# Autodesk Inventor assembly: Assembly
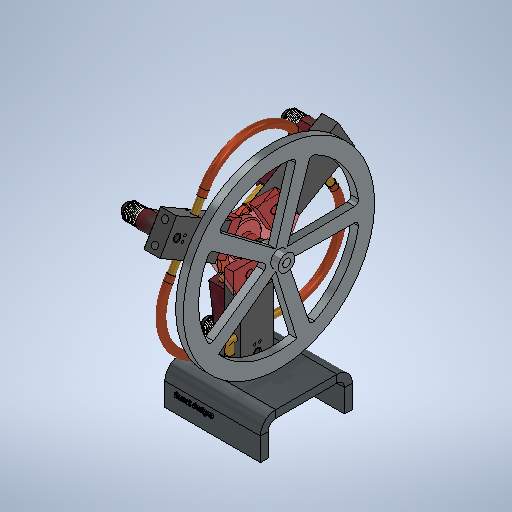
[picture p0: Inventor's stored thumbnail of the model, 512x512]
Saved by Autodesk Inventor 2025 (Build 290162010, 162A)
## iProperties
Created: 2024-06-06
Part Number: Assembly
Document SubType Name: Assembly
Designer: ffogue
Author: ffogue
## Documents named in this file (16)
- C:\Users\Fabri\Documents\Inventor\oscillatingEngine\Assembly.iam
- C:\Users\Fabri\Documents\Inventor\oscillatingEngine\support.ipt
- C:\Users\Fabri\Documents\Inventor\oscillatingEngine\base.ipt
- C:\Users\Fabri\Documents\Inventor\oscillatingEngine\adapter.ipt
- C:\Users\Fabri\Documents\Inventor\oscillatingEngine\divider.ipt
- C:\Users\Fabri\Documents\Inventor\oscillatingEngine\Tube.ipt
- C:\Users\Fabri\Documents\Inventor\oscillatingEngine\fitting.ipt
- C:\Users\Fabri\Documents\Inventor\oscillatingEngine\tube2.ipt
- C:\Users\Fabri\Documents\Inventor\oscillatingEngine\Plate.ipt
- C:\Users\Fabri\Documents\Inventor\oscillatingEngine\AdapterSupport.ipt
- C:\Users\Fabri\Documents\Inventor\oscillatingEngine\AdapterSupportAbove.ipt
- C:\Users\Fabri\Documents\Inventor\oscillatingEngine\handle.ipt
- C:\Users\Fabri\Documents\Inventor\oscillatingEngine\BromzeFitting.ipt
- C:\Users\Fabri\Documents\Inventor\oscillatingEngine\wheel.ipt
- C:\Users\Fabri\Documents\Inventor\oscillatingEngine\screw.ipt
- C:\Users\Fabri\Documents\Inventor\oscillatingEngine\Compress Spring12.ipt
## Components (29 placed, 15 different names)
1. support:1 — Insert:2, Insert:3, Mate:4, Insert:9, Mate:11, Insert:20
2. adapter:1 — Insert:2, Cylindrical:2, Mate:27, Insert:25
3. divider:1 — Insert:3, Mate:13
4. Tube:1 — Insert:13, Mate:13
5. fitting:1 — Insert:12, Mate:11
6. fitting:2 — Insert:11, Mate:10
7. fitting:3 — Insert:13, Mate:12
8. support:2 — Mate:5, Mate:8, Mate:9, Flush:2, Mate:10, Mate:15, Insert:17
9. support:3 — Mate:6, Mate:7, Flush:1, Mate:12, Mate:16, Insert:18
10. Plate:1 — Mate:4, Insert:9, Mate:5, Mate:6, Mate:7, Flush:1, Mate:8, Mate:9, Flush:2, Insert:19
11. tube2:1 — Insert:11, Insert:12
12. tube2:2 — Insert:15, Insert:16
13. fitting:4 — Insert:16, Mate:16
14. fitting:5 — Insert:15, Mate:15
15. adapter:2 — Insert:17, Cylindrical:3, Mate:25, Insert:24
16. adapter:3 — Insert:18, Cylindrical:1, Mate:26, Insert:23
17. AdapterSupport:1 — Mate:19, Cylindrical:2
18. AdapterSupportAbove:1 — Mate:20, Cylindrical:3
19. AdapterSupportAbove:2 — Mate:18, Cylindrical:1
20. handle:1 — Insert:19, Mate:18, Mate:19, Mate:20, Angle:1, Mate:21, Insert:21, Insert:22, Angle:2
21. base:1 — Insert:20
22. BromzeFitting:1 — Mate:21, Insert:21
23. wheel:1 — Insert:22, Angle:2
24. screw:1 — Mate:22, Flush:3, Mate:26, Insert:23
25. Compress Spring1:1 — Mate:22, Flush:3
26. screw:2 — Mate:27, Insert:25
27. Compress Spring1:2
28. screw:3 — Mate:25, Insert:24
29. Compress Spring1:3
## Relationships (49: Mate 22, Insert 17, Flush 5, CylindricalJoint 3, Angle 2)
- Insert:2: support:1 ↔ adapter:1
- Insert:3 (-9 mm): support:1 ↔ divider:1
- Mate:4: support:1 ↔ Plate:1
- Insert:9: support:1 ↔ Plate:1
- Mate:5: support:2 ↔ Plate:1
- Mate:6: support:3 ↔ Plate:1
- Mate:7: support:3 ↔ Plate:1
- Flush:1: support:3 ↔ Plate:1
- Mate:8: support:2 ↔ Plate:1
- Mate:9: support:2 ↔ Plate:1
- Flush:2: support:2 ↔ Plate:1
- Insert:11 (-2 mm): fitting:2 ↔ tube2:1
- Insert:12: fitting:1 ↔ tube2:1
- Mate:10: fitting:2 ↔ support:2
- Mate:11: support:1 ↔ fitting:1
- Insert:13: Tube:1 ↔ fitting:3
- Mate:12: fitting:3 ↔ support:3
- Mate:13: divider:1 ↔ Tube:1
- Insert:15: tube2:2 ↔ fitting:5
- Mate:15: support:2 ↔ fitting:5
- Insert:16: tube2:2 ↔ fitting:4
- Mate:16: support:3 ↔ fitting:4
- Insert:17: support:2 ↔ adapter:2
- Insert:18: support:3 ↔ adapter:3
- Insert:19 (-29 mm): Plate:1 ↔ handle:1
- Mate:18: AdapterSupportAbove:2 ↔ handle:1
- Cylindrical:1: adapter:3 ↔ AdapterSupportAbove:2
- Mate:19: AdapterSupport:1 ↔ handle:1
- Cylindrical:2: adapter:1 ↔ AdapterSupport:1
- Mate:20: AdapterSupportAbove:1 ↔ handle:1
- Cylindrical:3: adapter:2 ↔ AdapterSupportAbove:1
- Angle:1 (0 deg): handle:1
- Insert:20: support:1 ↔ base:1
- Mate:21: handle:1 ↔ BromzeFitting:1
- Insert:21 (-33 mm): handle:1 ↔ BromzeFitting:1
- Insert:22 (-18 mm): handle:1 ↔ wheel:1
- Mate:22: screw:1 ↔ Compress Spring1:1
- Flush:3: screw:1 ↔ Compress Spring1:1
- [Mate]: screw:2 ↔ Compress Spring1:2
- [Flush]: screw:2 ↔ Compress Spring1:2
- [Mate]: screw:3 ↔ Compress Spring1:3
- [Flush]: screw:3 ↔ Compress Spring1:3
- Mate:25: adapter:2 ↔ screw:3
- Mate:26: adapter:3 ↔ screw:1
- Mate:27: adapter:1 ↔ screw:2
- Insert:23 (-26 mm): adapter:3 ↔ screw:1
- Insert:24 (-26 mm): adapter:2 ↔ screw:3
- Insert:25 (-26 mm): adapter:1 ↔ screw:2
- Angle:2 (0 deg): handle:1 ↔ wheel:1
## Named parameters: d151_d149 = 0 mm, d152_d150 = 0 mm, d153_d149 = 0 mm, d154_d150 = 0 mm
